# Autodesk Inventor assembly: Wing_tip
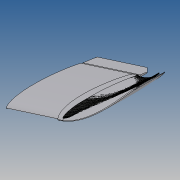
[picture p0: Inventor's stored thumbnail of the model, 180x180]
Saved by Autodesk Inventor 2019.4 (Build 234330000, 330)
## iProperties
Part Number: Wing_tip
Document SubType Name: Assembly
Designer: Admin
Mass: 10564 g
Surface Area: 1637.39 cm^2
Volume: 1344.02 cm^3
Density: 7.86 g/cm^3
Author: Admin
Revision: -
VAULT_Status: in Bearbeitung
Gewicht: 10,564 kg
InventorVersion: 2019.4
## Documents named in this file (5)
- C:\Users\tonn\Documents\GitHub\CAD_Elements\CAD\bashy\Wing_tip.iam
- Norm.iam
- C:\Users\tonn\Documents\GitHub\CAD_Elements\CAD\bashy\Wingtip.ipt
- C:\Users\tonn\Documents\GitHub\CAD_Elements\CAD\bashy\Wing_airfoil.ipt
- C:\Users\tonn\Downloads\recon_50_shorts.ipt
## Components (3 placed, 3 different names)
1. WING_AIRFOIL_WINGTIP--IPT:1 — Fluchtend:1, Fluchtend:2, Passend:4
2. WING_AIRFOIL_WING_AIRFOIL--IPT:1 — Fluchtend:1, Fluchtend:2, Passend:2, Passend:3, Passend:4
3. recon_50_shorts:1 — Passend:2, Passend:3
## Relationships (5: Mate 3, Flush 2)
- Fluchtend:1 [Flush]: WING_AIRFOIL_WINGTIP--IPT:1 ↔ WING_AIRFOIL_WING_AIRFOIL--IPT:1
- Fluchtend:2 [Flush]: WING_AIRFOIL_WINGTIP--IPT:1 ↔ WING_AIRFOIL_WING_AIRFOIL--IPT:1
- Passend:2 [Mate] (66 mm): WING_AIRFOIL_WING_AIRFOIL--IPT:1 ↔ recon_50_shorts:1
- Passend:3 [Mate] (1 mm): WING_AIRFOIL_WING_AIRFOIL--IPT:1 ↔ recon_50_shorts:1
- Passend:4 [Mate] (1 mm): WING_AIRFOIL_WINGTIP--IPT:1 ↔ WING_AIRFOIL_WING_AIRFOIL--IPT:1
## Named parameters: Gewicht = 10.564
note: some values were not read from the file. Shown as the stored number, unit unknown: "Gewicht".
